# Autodesk Inventor assembly: 基本構造
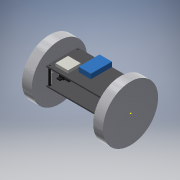
[picture p0: Inventor's stored thumbnail of the model, 180x180]
Saved by Autodesk Inventor 2017 (Build 210142000, 142)
## iProperties
Part Number: 基本構造
Material: 一般
Document SubType Name: Assembly
Designer: HISAAKI
Author: HISAAKI
## Documents named in this file (11)
- C:\Users\HISAAKI\Documents\LYNCS\CanSat\2017種子島\cansat-structure\基本構造.iam
- C:\Users\HISAAKI\Documents\LYNCS\CanSat\2017種子島\cansat-structure\基本板.ipt
- C:\Users\HISAAKI\Documents\LYNCS\CanSat\2017種子島\cansat-structure\既成部品\ブラケット.ipt
- C:\Users\HISAAKI\Documents\LYNCS\CanSat\2017種子島\cansat-structure\既成部品\モータ.ipt
- C:\Users\HISAAKI\Documents\LYNCS\CanSat\2017種子島\cansat-structure\ハブver1.1.ipt
- C:\Users\HISAAKI\Documents\LYNCS\CanSat\2017種子島\cansat-structure\タイヤスポンジ部分.ipt
- C:\Users\HISAAKI\Documents\LYNCS\CanSat\2017種子島\cansat-structure\既成部品\リポ電池.ipt
- C:\Users\HISAAKI\Documents\LYNCS\CanSat\2017種子島\cansat-structure\基本板上.ipt
- C:\Users\HISAAKI\Documents\LYNCS\CanSat\2017種子島\cansat-structure\既成部品\mbed.ipt
- C:\Users\HISAAKI\Documents\LYNCS\CanSat\2017種子島\cansat-structure\既成部品\スペーサ.ipt
- C:\Users\HISAAKI\Documents\LYNCS\CanSat\2017種子島\cansat-structure\既成部品\GPSユニット.ipt
## Components (17 placed, 10 different names)
1. 基本板:1 — フラッシュ:1, フラッシュ:2, メイト:19, メイト:20, メイト:21, メイト:23, メイト:24, メイト:25, メイト:26, メイト:27, メイト:28, メイト:29, メイト:30, フラッシュ:4, フラッシュ:6, メイト:35, メイト:36, メイト:37, メイト:38, メイト:39, メイト:40
2. モータ:1 — フラッシュ:2, メイト:13, メイト:14, メイト:41, メイト:43
3. モータ:2 — フラッシュ:1, メイト:11, メイト:12, メイト:42, メイト:44
4. ハブver1.1:1 — メイト:11, メイト:12, メイト:17, メイト:18
5. ハブver1.1:2 — メイト:13, メイト:14, メイト:15, メイト:16
6. タイヤスポンジ部分:1 — メイト:15, メイト:16
7. タイヤスポンジ部分:2 — メイト:17, メイト:18
8. リポ電池:1 — メイト:19, フラッシュ:4, フラッシュ:6
9. 基本板上:1 — メイト:20, メイト:21, メイト:22, フラッシュ:3, メイト:31, メイト:32, メイト:33, フラッシュ:5
10. mbed:1 — メイト:22, フラッシュ:3, メイト:33, メイト:34
11. スペーサ:1 — メイト:23, メイト:29
12. スペーサ:2 — メイト:25, メイト:28
13. スペーサ:3 — メイト:24, メイト:30, メイト:31
14. スペーサ:4 — メイト:26, メイト:27
15. GPSユニット:1 — メイト:32, メイト:34, フラッシュ:5
16. ブラケット:1 — メイト:35, メイト:36, メイト:37, メイト:41, メイト:43
17. ブラケット:2 — メイト:38, メイト:39, メイト:40, メイト:42, メイト:44
## Relationships (40: Mate 34, Flush 6)
- フラッシュ:1 [Flush]: 基本板:1 ↔ モータ:2
- フラッシュ:2 [Flush]: 基本板:1 ↔ モータ:1
- メイト:11 [Mate]: モータ:2 ↔ ハブver1.1:1
- メイト:12 [Mate]: モータ:2 ↔ ハブver1.1:1
- メイト:13 [Mate]: モータ:1 ↔ ハブver1.1:2
- メイト:14 [Mate]: モータ:1 ↔ ハブver1.1:2
- メイト:15 [Mate]: ハブver1.1:2 ↔ タイヤスポンジ部分:1
- メイト:16 [Mate]: ハブver1.1:2 ↔ タイヤスポンジ部分:1
- メイト:17 [Mate]: ハブver1.1:1 ↔ タイヤスポンジ部分:2
- メイト:18 [Mate]: ハブver1.1:1 ↔ タイヤスポンジ部分:2
- メイト:19 [Mate]: 基本板:1 ↔ リポ電池:1
- メイト:20 [Mate]: 基本板:1 ↔ 基本板上:1
- メイト:21 [Mate]: 基本板:1 ↔ 基本板上:1
- メイト:22 [Mate]: 基本板上:1 ↔ mbed:1
- フラッシュ:3 [Flush]: 基本板上:1 ↔ mbed:1
- メイト:23 [Mate]: 基本板:1 ↔ スペーサ:1
- メイト:24 [Mate]: 基本板:1 ↔ スペーサ:3
- メイト:25 [Mate]: 基本板:1 ↔ スペーサ:2
- メイト:26 [Mate]: 基本板:1 ↔ スペーサ:4
- メイト:27 [Mate]: 基本板:1 ↔ スペーサ:4
- メイト:28 [Mate]: 基本板:1 ↔ スペーサ:2
- メイト:29 [Mate]: 基本板:1 ↔ スペーサ:1
- メイト:30 [Mate]: 基本板:1 ↔ スペーサ:3
- メイト:31 [Mate]: 基本板上:1 ↔ スペーサ:3
- メイト:32 [Mate]: 基本板上:1 ↔ GPSユニット:1
- フラッシュ:4 [Flush] (40 mm): 基本板:1 ↔ リポ電池:1
- メイト:33 [Mate] (55.3 mm): 基本板上:1 ↔ mbed:1
- メイト:34 [Mate] (10 mm): mbed:1 ↔ GPSユニット:1
- フラッシュ:5 [Flush] (10 mm): 基本板上:1 ↔ GPSユニット:1
- フラッシュ:6 [Flush] (36 mm): 基本板:1 ↔ リポ電池:1
- メイト:35 [Mate]: 基本板:1 ↔ ブラケット:1
- メイト:36 [Mate]: 基本板:1 ↔ ブラケット:1
- メイト:37 [Mate]: 基本板:1 ↔ ブラケット:1
- メイト:38 [Mate]: 基本板:1 ↔ ブラケット:2
- メイト:39 [Mate]: 基本板:1 ↔ ブラケット:2
- メイト:40 [Mate]: 基本板:1 ↔ ブラケット:2
- メイト:41 [Mate]: モータ:1 ↔ ブラケット:1
- メイト:42 [Mate]: モータ:2 ↔ ブラケット:2
- メイト:43 [Mate]: モータ:1 ↔ ブラケット:1
- メイト:44 [Mate]: モータ:2 ↔ ブラケット:2
## Named parameters: sa_0 = -6000, sa_1 = -3.93e-11, sa_2 = -1.3e-12
note: some values were not read from the file. Shown as the stored number, unit unknown: "sa_0", "sa_1", "sa_2".
